# Autodesk Inventor assembly: Wine Rack and Light Shelf Assembly
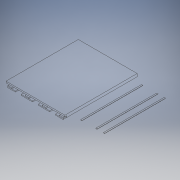
[picture p0: Inventor's stored thumbnail of the model, 180x180]
Saved by Autodesk Inventor 2016 (Build 200138000, 138)
## iProperties
Created: 2017-11-04
Part Number: Wine Rack and Light Shelf Assembly
Document SubType Name: Assembly
Designer: mathaetaes
Author: mathaetaes
## Documents named in this file (4)
- E:\Projects\3D Printer\printer projects\My Designs\Bar Cabinet\Wine Rack and Light Shelf Assembly.iam
- E:\Projects\3D Printer\printer projects\My Designs\Bar Cabinet\Horizontal Shelf with Lights.ipt
- E:\Projects\3D Printer\printer projects\My Designs\Bar Cabinet\Wine Glass Rack Full Assembly.iam
- E:\Projects\3D Printer\printer projects\My Designs\Bar Cabinet\LED light strip.ipt
## Components (5 placed, 3 different names)
1. Horizontal Shelf with Lights:1 — Flush:1, Mate:1, Flush:2
2. Wine Glass Rack Full Assembly:1 [sub-assembly] — Flush:1, Mate:1, Flush:2
3. LED light strip:1
4. LED light strip:2
5. LED light strip:3
## Relationships (3: Flush 2, Mate 1)
- Flush:1: Horizontal Shelf with Lights:1 ↔ Wine Glass Rack Full Assembly:1
- Mate:1: Horizontal Shelf with Lights:1 ↔ Wine Glass Rack Full Assembly:1
- Flush:2 (12.7 mm): Horizontal Shelf with Lights:1 ↔ Wine Glass Rack Full Assembly:1
